# Autodesk Inventor assembly: ultima gamba
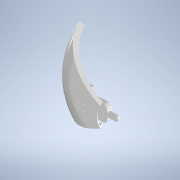
[picture p0: Inventor's stored thumbnail of the model, 180x180]
Saved by Autodesk Inventor 2020.2 (Build 242310000, 310)
## iProperties
Created: 2020-05-09
Part Number: ultima gamba
Document SubType Name: Assembly
Designer: mazzo
Author: mazzo
## Documents named in this file (5)
- C:\Users\User\Desktop\Progetto Meccanica dei Robot\assembled in urdf\nuovi\shell.iam
- C:\Users\User\Desktop\Progetto Meccanica dei Robot\meccanica\parti autodesk\V3turbo\gamba3.3.ipt
- C:\Users\User\Desktop\Progetto Meccanica dei Robot\meccanica\parti autodesk\V3turbo\bottom_shell.ipt
- C:\Users\User\Desktop\Progetto Meccanica dei Robot\meccanica\parti autodesk\V3turbo\end_effector_semplificato.ipt
- C:\Users\User\Desktop\Progetto Meccanica dei Robot\meccanica\parti autodesk\V3turbo\Motore1.ipt
## Components (4 placed, 4 different names)
1. gamba3.3:1 — Cilindrico:1, Allineato:1, Rotazionale:1, Cilindrico:2, Coincidente:1, Angolo:1, Rotazionale:2, Cilindrico:3
2. bottom_shell:1 — Rotazionale:1, Cilindrico:2
3. end_effector_semplificato:1 — Cilindrico:1, Allineato:1, Coincidente:1, Coincidente:2, Tangente:1
4. Motore1:1 — Rotazionale:2, Cilindrico:3
## Relationships (11: CylindricalJoint 3, Mate 3, RevoluteJoint 2, Flush 1, Tangent 1, Angle 1)
- Cilindrico:1 [CylindricalJoint]: gamba3.3:1 ↔ end_effector_semplificato:1
- Allineato:1 [Flush]: gamba3.3:1 ↔ end_effector_semplificato:1
- Rotazionale:1 [RevoluteJoint]: gamba3.3:1 ↔ bottom_shell:1
- Cilindrico:2 [CylindricalJoint]: gamba3.3:1 ↔ bottom_shell:1
- Coincidente:1 [Mate]: gamba3.3:1 ↔ end_effector_semplificato:1
- Coincidente:2 [Mate]: end_effector_semplificato:1
- Coincidente:3 [Mate]
- Tangente:1: end_effector_semplificato:1
- Angolo:1 [Angle] (0 deg): gamba3.3:1
- Rotazionale:2 [RevoluteJoint]: gamba3.3:1 ↔ Motore1:1
- Cilindrico:3 [CylindricalJoint]: gamba3.3:1 ↔ Motore1:1
